# Autodesk Inventor assembly: Spider
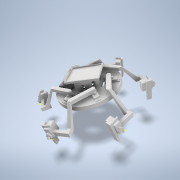
[picture p0: Inventor's stored thumbnail of the model, 180x180]
Saved by Autodesk Inventor 2022 (Build 260153000, 153)
## iProperties
Created: 2023-07-22
Part Number: Spider
Document SubType Name: Assembly
Designer: Eric Cao
Author: Eric Cao
## Documents named in this file (5)
- D:\CAD Practice\SpiderBot\Assemblies\Spider.iam
- D:\CAD Practice\SpiderBot\Drawings\Base.ipt
- D:\CAD Practice\SpiderBot\Drawings\Servo Motor.ipt
- D:\CAD Practice\SpiderBot\Drawings\leg.ipt
- D:\CAD Practice\SpiderBot\Drawings\connector.ipt
## Components (25 placed, 4 different names)
1. Base:1 — Rigid:2
2. Servo Motor:11 — Rigid:2
3. Servo Motor:23
4. Servo Motor:24
5. Servo Motor:25
6. Servo Motor:26
7. Servo Motor:27 — Rotational:1
8. connector:11 — Rotational:1, Rotational:2
9. Servo Motor:10 — Rigid:1, Rotational:2
10. leg:1 — Rigid:1
11. connector:12
12. Servo Motor:28
13. leg:2
14. connector:13
15. Servo Motor:29
16. leg:3
17. connector:14
18. Servo Motor:30
19. leg:4
20. connector:15
21. Servo Motor:31
22. leg:5
23. connector:16
24. Servo Motor:32
25. leg:6
## Component patterns: (6 elements, first: Servo Motor:11), (6 elements, first: connector:11 + Servo Motor:10 + leg:1)
## Relationships (4: WeldJoint 2, RevoluteJoint 2)
- Rigid:1 [WeldJoint]: Servo Motor:10 ↔ leg:1
- Rigid:2 [WeldJoint]: Base:1 ↔ Servo Motor:11
- Rotational:1 [RevoluteJoint]: Servo Motor:27 ↔ connector:11
- Rotational:2 [RevoluteJoint]: connector:11 ↔ Servo Motor:10
